# Autodesk Inventor assembly: 0001_ASS_Hop_so
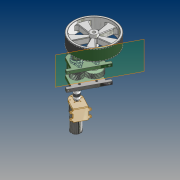
[picture p0: Inventor's stored thumbnail of the model, 180x180]
Saved by Autodesk Inventor 2021 (Build 250183000, 183)
## iProperties
Created: 2024-04-07
Part Number: 0001_ASS_Hop_so
Document SubType Name: Assembly
Designer: Admin
Mass: 1909.58 g
Surface Area: 1802.26 cm^2
Volume: 462.406 cm^3
Density: 4.12966 g/cm^3
Author: Admin
## Documents named in this file (12)
- C:\Users\Admin\Desktop\DO_AN_TOT_NGHIEP_2024\Mechanical\Design_in_3D\Version_1\0001_ASS_Hop_so.iam
- C:\Users\Admin\Desktop\DO_AN_TOT_NGHIEP_2024\Mechanical\Design_in_3D\Library\Banh_rang\Final_Rang_Lon.ipt
- C:\Users\Admin\Desktop\DO_AN_TOT_NGHIEP_2024\Mechanical\Design_in_3D\Library\Banh_rang\Final_Rang_Nho.ipt
- C:\Users\Admin\Desktop\DO_AN_TOT_NGHIEP_2024\Mechanical\Design_in_3D\Version_1\22_Hop_so_ngang.ipt
- C:\Users\Admin\Desktop\DO_AN_TOT_NGHIEP_2024\Mechanical\Design_in_3D\Library\kfl000-bearing-unit-10mm-1.snapshot.3\KFL000 bearing unit 10mm.iam
- C:\Users\Admin\Desktop\DO_AN_TOT_NGHIEP_2024\Mechanical\Design_in_3D\Library\08_Ga_dong_co_02.ipt
- C:\Users\Admin\Desktop\DO_AN_TOT_NGHIEP_2024\Mechanical\Design_in_3D\Library\DC_Servo_JGB37-520.iam
- C:\Users\Admin\Desktop\DO_AN_TOT_NGHIEP_2024\Mechanical\Design_in_3D\Library\kh-p-n-i-m-m-2.snapshot.1\khop-noi-mem.ipt
- C:\Users\Admin\Desktop\DO_AN_TOT_NGHIEP_2024\Mechanical\Design_in_3D\Version_1\01_Truc_02.ipt
- C:\Users\Admin\Desktop\DO_AN_TOT_NGHIEP_2024\Mechanical\Design_in_3D\Version_1\02_Truc_02.ipt
- C:\Users\Admin\Desktop\DO_AN_TOT_NGHIEP_2024\Mechanical\Design_in_3D\Version_1\23_Nap_hop_so_ngang.ipt
- C:\Users\Admin\Desktop\DO_AN_TOT_NGHIEP_2024\Mechanical\Design_in_3D\Library\Banh_xe.iam
## Components (15 placed, 11 different names)
1. 22_Hop_so_ngang:1 — Flush:2, Mate:4, Mate:8, Mate:9, Mate:10, Angle:1, Mate:28, Angle:6, Angle:7
2. 22_Hop_so_ngang:2 — Flush:2, Mate:6, Mate:7, Mate:11, Mate:12, Angle:2, Angle:3, Flush:3, Mate:24, Flush:6, Mate:25, Mate:29
3. KFL000 bearing unit 10mm:1 [sub-assembly] — Mate:4, Mate:10, Angle:4, Mate:30
4. KFL000 bearing unit 10mm:2 [sub-assembly] — Mate:7, Mate:11, Angle:3, Mate:17, Mate:20
5. KFL000 bearing unit 10mm:3 [sub-assembly] — Mate:6, Mate:12, Angle:2, Insert:1
6. KFL000 bearing unit 10mm:4 [sub-assembly] — Mate:8, Mate:9, Angle:1, Angle:4, Flush:4
7. 08_Ga_dong_co_02:1 — Mate:15, Angle:5, Mate:16, Flush:3
8. DC_Servo_JGB37-520:1 [sub-assembly] — Mate:15, Angle:5, Mate:16, Mate:17, Mate:19, Mate:22
9. khop-noi-mem:1 — Mate:19, Mate:21, Mate:22
10. 01_Truc_02:1 — Mate:20, Flush:4, Mate:21, Mate:27
11. 02_Truc_02:1 — Insert:1, Mate:26, Mate:30, Insert:2
12. 23_Nap_hop_so_ngang:1 — Mate:24, Flush:6, Mate:25
13. Spur Gear1:2 — Mate:27, Flush:7
14. Spur Gear2:2 — Mate:26, Flush:7, Mate:28, Mate:29
15. Banh_xe:1 [sub-assembly] — Insert:2, Tangent:1
## Relationships (38: Mate 23, Angle 7, Flush 5, Insert 2, Tangent 1)
- Flush:2: 22_Hop_so_ngang:1 ↔ 22_Hop_so_ngang:2
- Mate:4: 22_Hop_so_ngang:1 ↔ KFL000 bearing unit 10mm:1
- Mate:6: 22_Hop_so_ngang:2 ↔ KFL000 bearing unit 10mm:3
- Mate:7: 22_Hop_so_ngang:2 ↔ KFL000 bearing unit 10mm:2
- Mate:8: 22_Hop_so_ngang:1 ↔ KFL000 bearing unit 10mm:4
- Mate:9: 22_Hop_so_ngang:1 ↔ KFL000 bearing unit 10mm:4
- Mate:10: 22_Hop_so_ngang:1 ↔ KFL000 bearing unit 10mm:1
- Mate:11: 22_Hop_so_ngang:2 ↔ KFL000 bearing unit 10mm:2
- Mate:12: 22_Hop_so_ngang:2 ↔ KFL000 bearing unit 10mm:3
- Angle:1 (0 deg): 22_Hop_so_ngang:1 ↔ KFL000 bearing unit 10mm:4
- Angle:2 (0 deg): 22_Hop_so_ngang:2 ↔ KFL000 bearing unit 10mm:3
- Angle:3 (0 deg): 22_Hop_so_ngang:2 ↔ KFL000 bearing unit 10mm:2
- Angle:4 (180 deg): KFL000 bearing unit 10mm:1 ↔ KFL000 bearing unit 10mm:4
- Mate:15: 08_Ga_dong_co_02:1 ↔ DC_Servo_JGB37-520:1
- Angle:5 (180 deg): 08_Ga_dong_co_02:1 ↔ DC_Servo_JGB37-520:1
- Mate:16: 08_Ga_dong_co_02:1 ↔ DC_Servo_JGB37-520:1
- Mate:17: KFL000 bearing unit 10mm:2 ↔ DC_Servo_JGB37-520:1
- Flush:3: 22_Hop_so_ngang:2 ↔ 08_Ga_dong_co_02:1
- [Mate]: khop-noi-mem:1 ↔ 01_Truc_02:1
- Mate:19: DC_Servo_JGB37-520:1 ↔ khop-noi-mem:1
- Mate:20: KFL000 bearing unit 10mm:2 ↔ 01_Truc_02:1
- Flush:4: KFL000 bearing unit 10mm:4 ↔ 01_Truc_02:1
- Mate:21 (-7 mm): khop-noi-mem:1 ↔ 01_Truc_02:1
- Mate:22 (-7 mm): DC_Servo_JGB37-520:1 ↔ khop-noi-mem:1
- Insert:1: KFL000 bearing unit 10mm:3 ↔ 02_Truc_02:1
- Mate:24: 22_Hop_so_ngang:2 ↔ 23_Nap_hop_so_ngang:1
- Flush:6: 22_Hop_so_ngang:2 ↔ 23_Nap_hop_so_ngang:1
- Mate:25: 22_Hop_so_ngang:2 ↔ 23_Nap_hop_so_ngang:1
- Mate:26: 02_Truc_02:1 ↔ Spur Gear2:2
- Mate:27: 01_Truc_02:1 ↔ Spur Gear1:2
- Flush:7: Spur Gear1:2 ↔ Spur Gear2:2
- Mate:28 (10 mm): 22_Hop_so_ngang:1 ↔ Spur Gear2:2
- Mate:29 (10 mm): 22_Hop_so_ngang:2 ↔ Spur Gear2:2
- Mate:30: KFL000 bearing unit 10mm:1 ↔ 02_Truc_02:1
- Insert:2 (-10 mm): 02_Truc_02:1 ↔ Banh_xe:1
- Angle:6 (0 deg): 22_Hop_so_ngang:1
- Tangent:1: Banh_xe:1
- Angle:7 (180 deg): 22_Hop_so_ngang:1
